# Autodesk Inventor assembly: Assembly1
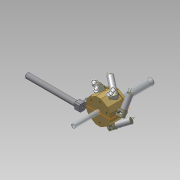
[picture p0: Inventor's stored thumbnail of the model, 180x180]
Saved by Autodesk Inventor 2014 (Build 180170000, 170)
## iProperties
Created: 2015-05-11
Part Number: Assembly1
Document SubType Name: Assembly
Designer: Admin
Author: Admin
## Documents named in this file (11)
- D:\autodesk_files\3+2_ch_steady\Assembly1.iam
- D:\autodesk_files\3+2_ch_steady\body.ipt
- D:\autodesk_files\3+2_ch_steady\nozzle_small.ipt
- D:\autodesk_files\3+2_ch_steady\nozzle_big.ipt
- D:\autodesk_files\3+2_ch_steady\tube.ipt
- D:\autodesk_files\3+2_ch_steady\tube_long.ipt
- D:\autodesk_files\3+2_ch_steady\holder.ipt
- D:\autodesk_files\3+2_ch_steady\rod.ipt
- D:\autodesk_files\3+2_ch_steady\valve.ipt
- C:\Users\Admin\Documents\Inventor\Content Center Files\R2014\en-US\ANSI B18.3.1M(6)\ANSI B18.3.1M - M2x0,4 x 6(1).ipt
- C:\Users\Admin\Documents\Inventor\Content Center Files\R2014\en-US\ANSI B18.3.1M(6)\ANSI B18.3.1M - M4x0,7 x 10(1).ipt
## Components (24 placed, 10 different names)
1. body:1 — Insert:1, Insert:2, Insert:5, Insert:7, Insert:8, Insert:9, Insert:10, Insert:11, Insert:12, Insert:13, Insert:14, Insert:15
2. nozzle_small:1 — Insert:1, Insert:3
3. nozzle_big:1 — Insert:2, Insert:4
4. tube:1 — Insert:3
5. tube_long:1 — Insert:4
6. holder:1 — Insert:5, Insert:6, Insert:26, Insert:27
7. rod:1 — Insert:6
8. valve:1 — Insert:7, Insert:8, Insert:18, Insert:19
9. valve:2 — Insert:9, Insert:16, Insert:17
10. valve:3 — Insert:10, Insert:11, Insert:24, Insert:25
11. valve:4 — Insert:12, Insert:13, Insert:20, Insert:21
12. valve:5 — Insert:14, Insert:15, Insert:22, Insert:23
13. Forged Socket Head Cap Screw - Metric M2x0,4 x 6:1 — Insert:16
14. Forged Socket Head Cap Screw - Metric M2x0,4 x 6:2 — Insert:19
15. Forged Socket Head Cap Screw - Metric M2x0,4 x 6:3 — Insert:23
16. Forged Socket Head Cap Screw - Metric M2x0,4 x 6:4 — Insert:24
17. Forged Socket Head Cap Screw - Metric M2x0,4 x 6:5 — Insert:25
18. Forged Socket Head Cap Screw - Metric M2x0,4 x 6:6 — Insert:17
19. Forged Socket Head Cap Screw - Metric M2x0,4 x 6:7 — Insert:18
20. Forged Socket Head Cap Screw - Metric M2x0,4 x 6:8 — Insert:20
21. Forged Socket Head Cap Screw - Metric M2x0,4 x 6:9 — Insert:22
22. Forged Socket Head Cap Screw - Metric M2x0,4 x 6:10 — Insert:21
23. Forged Socket Head Cap Screw - Metric M4x0,7 x 10:1 — Insert:26
24. Forged Socket Head Cap Screw - Metric M4x0,7 x 10:2 — Insert:27
## Relationships (27: Insert 27)
- Insert:1: body:1 ↔ nozzle_small:1
- Insert:2: body:1 ↔ nozzle_big:1
- Insert:3: nozzle_small:1 ↔ tube:1
- Insert:4: nozzle_big:1 ↔ tube_long:1
- Insert:5: body:1 ↔ holder:1
- Insert:6: holder:1 ↔ rod:1
- Insert:7: body:1 ↔ valve:1
- Insert:8: body:1 ↔ valve:1
- Insert:9: body:1 ↔ valve:2
- Insert:10: body:1 ↔ valve:3
- Insert:11: body:1 ↔ valve:3
- Insert:12: body:1 ↔ valve:4
- Insert:13: body:1 ↔ valve:4
- Insert:14: body:1 ↔ valve:5
- Insert:15: body:1 ↔ valve:5
- Insert:16: valve:2 ↔ Forged Socket Head Cap Screw - Metric M2x0,4 x 6:1
- Insert:17: valve:2 ↔ Forged Socket Head Cap Screw - Metric M2x0,4 x 6:6
- Insert:18: valve:1 ↔ Forged Socket Head Cap Screw - Metric M2x0,4 x 6:7
- Insert:19: valve:1 ↔ Forged Socket Head Cap Screw - Metric M2x0,4 x 6:2
- Insert:20: valve:4 ↔ Forged Socket Head Cap Screw - Metric M2x0,4 x 6:8
- Insert:21: valve:4 ↔ Forged Socket Head Cap Screw - Metric M2x0,4 x 6:10
- Insert:22: valve:5 ↔ Forged Socket Head Cap Screw - Metric M2x0,4 x 6:9
- Insert:23: valve:5 ↔ Forged Socket Head Cap Screw - Metric M2x0,4 x 6:3
- Insert:24: valve:3 ↔ Forged Socket Head Cap Screw - Metric M2x0,4 x 6:4
- Insert:25: valve:3 ↔ Forged Socket Head Cap Screw - Metric M2x0,4 x 6:5
- Insert:26: holder:1 ↔ Forged Socket Head Cap Screw - Metric M4x0,7 x 10:1
- Insert:27: holder:1 ↔ Forged Socket Head Cap Screw - Metric M4x0,7 x 10:2
